# Autodesk Inventor assembly: korp
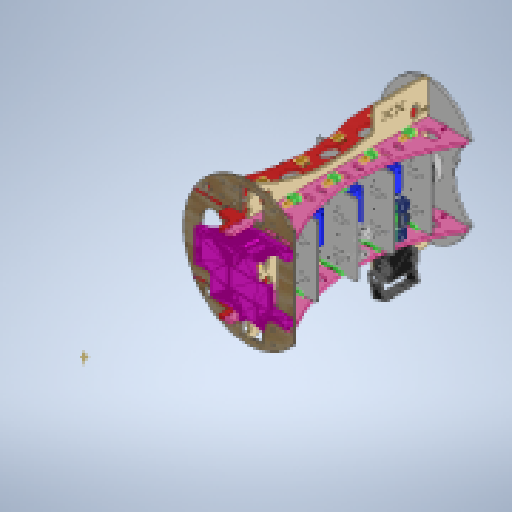
[picture p0: Inventor's stored thumbnail of the model, 512x512]
Saved by Autodesk Inventor 2023.1 (Build 271208000, 208)
## iProperties
Created: 2023-03-13
Part Number: korp
Document SubType Name: Assembly
Designer: User
Author: User
## Documents named in this file (23)
- C:\Users\DELL\reposGitHub\Cheburashka\Cheburashka_construction\korpus\korp.iam
- C:\Users\DELL\reposGitHub\Cheburashka\Cheburashka_construction\korpus\нижний эллипс тела.ipt
- C:\Users\DELL\reposGitHub\Cheburashka\Cheburashka_construction\korpus\грань тела.ipt
- C:\Users\DELL\reposGitHub\Cheburashka\Cheburashka_construction\korpus\Servo.ipt
- C:\Users\DELL\reposGitHub\Cheburashka\Cheburashka_construction\platform\KRAVT_holder_2 (1).ipt
- C:\Users\DELL\reposGitHub\Cheburashka\Cheburashka_construction\korpus\ребро.ipt
- C:\Users\DELL\reposGitHub\Cheburashka\Cheburashka_construction\korpus\ребро_MIR.ipt
- C:\Users\DELL\reposGitHub\Cheburashka\Cheburashka_construction\korpus\креп.ipt
- C:\Users\DELL\reposGitHub\Cheburashka\Cheburashka_construction\korpus\ребро0.5.ipt
- C:\Users\DELL\reposGitHub\Cheburashka\Cheburashka_construction\korpus\стабилизатор.ipt
- C:\Users\DELL\reposGitHub\Cheburashka\Cheburashka_construction\korpus\ограничитель.ipt
- C:\Users\DELL\reposGitHub\Cheburashka\Cheburashka_construction\korpus\ребро0.5_MIR3.ipt
- C:\Users\DELL\reposGitHub\Cheburashka\Cheburashka_construction\korpus\фанера.ipt
- C:\Users\DELL\reposGitHub\Cheburashka\Cheburashka_construction\korpus\ограничитель_MIR.ipt
- C:\Users\DELL\reposGitHub\Cheburashka\Cheburashka_construction\korpus\палка.ipt
- C:\Users\DELL\reposGitHub\Cheburashka\Cheburashka_construction\korpus\креп_MIR2.ipt
- C:\Users\DELL\reposGitHub\Cheburashka\Cheburashka_construction\korpus\палка_MIR.ipt
- C:\Users\DELL\reposGitHub\Cheburashka\Cheburashka_construction\korpus\raspberry-pi-4-model-b-1.snapshot.3\Raspberry Pi 4 Model B.iam
- C:\Users\DELL\reposGitHub\Cheburashka\Cheburashka_construction\korpus\arduino-mega-2650-1.snapshot.2\arduino MEGA2650.iam
- C:\Users\DELL\reposGitHub\Cheburashka\Cheburashka_construction\korpus\acc2.ipt
- C:\Users\DELL\reposGitHub\Cheburashka\Cheburashka_construction\korpus\acc1.ipt
- C:\Users\DELL\reposGitHub\Cheburashka\Cheburashka_construction\face\лицо\креп_сервы.ipt
- C:\Users\DELL\reposGitHub\Cheburashka\Cheburashka_construction\korpus\turn.iam
## Components (54 placed, 22 different names)
1. нижний эллипс тела:1 — Совмещение:100, Совмещение:121, Совмещение:139, Совмещение:140, Совмещение:209, Совмещение:210
2. грань тела:1 — Совмещение:209, Совмещение:210, Совмещение:211, Совмещение:214, Совмещение:224, Совмещение:225, Совмещение:229, Совмещение:308
3. KRAVT_holder_2 (1):1 — Совмещение:100
4. ребро:1 — Совмещение:184, Совмещение:264, Совмещение:307
5. ребро_MIR:1 — Совмещение:122, Совмещение:188, Совмещение:204, Совмещение:305
6. креп:1 — Совмещение:159, Совмещение:166, Совмещение:221, Совмещение:222
7. креп:2 — Совмещение:164, Совмещение:165
8. креп:3 — Совмещение:162, Совмещение:163
9. креп:4 — Совмещение:160, Совмещение:161, Совмещение:219, Совмещение:220
10. креп:5 — Совмещение:167, Совмещение:168
11. креп:6 — Совмещение:169, Совмещение:170, Совмещение:183, Совмещение:217, Совмещение:218
12. креп:7 — Совмещение:261, Совмещение:262, Совмещение:265, Совмещение:266
13. креп:8 — Совмещение:171, Совмещение:172
14. ребро0.5:1 — Совмещение:121, Совмещение:122, Совмещение:126, Совмещение:128, Совмещение:129, Совмещение:130, Совмещение:132, Совмещение:133, Совмещение:135, Совмещение:136, Совмещение:138, Совмещение:186, Совмещение:187, Совмещение:189, Совмещение:190, Совмещение:191, Совмещение:192, Совмещение:193, Совмещение:194, Совмещение:195, Совмещение:196, Совмещение:197, Совмещение:198, Совмещение:199, Совмещение:200, Совмещение:201, Совмещение:202
15. стабилизатор:1
16. ребро0.5_MIR3:1 — Совмещение:139, Совмещение:140, Совмещение:159, Совмещение:160, Совмещение:161, Совмещение:162, Совмещение:163, Совмещение:164, Совмещение:165, Совмещение:166, Совмещение:167, Совмещение:168, Совмещение:169, Совмещение:170, Совмещение:171, Совмещение:172, Совмещение:261, Совмещение:262
17. ограничитель:1 — Совмещение:126, Совмещение:128, Совмещение:129
18. ограничитель:2 — Совмещение:130, Совмещение:132
19. ограничитель:3 — Совмещение:133, Совмещение:135
20. ограничитель:4 — Совмещение:136, Совмещение:138
21. фанера:1 — Совмещение:305, Совмещение:306
22. ограничитель_MIR:1
23. ограничитель_MIR:2
24. ограничитель_MIR:3
25. ограничитель_MIR:4
26. палка:1 — Совмещение:264, Совмещение:265, Совмещение:266
27. креп_MIR2:1 — Совмещение:199, Совмещение:200, Совмещение:203, Совмещение:303, Совмещение:304
28. креп_MIR2:2 — Совмещение:201, Совмещение:202
29. креп_MIR2:3 — Совмещение:197, Совмещение:198
30. креп_MIR2:4 — Совмещение:185, Совмещение:186, Совмещение:187, Совмещение:301, Совмещение:302
31. креп_MIR2:5 — Совмещение:195, Совмещение:196
32. креп_MIR2:6 — Совмещение:189, Совмещение:190, Совмещение:299, Совмещение:300
33. креп_MIR2:7 — Совмещение:180, Совмещение:181, Совмещение:182, Совмещение:191, Совмещение:192, Совмещение:306
34. креп_MIR2:8 — Совмещение:193, Совмещение:194
35. палка_MIR:1 — Совмещение:180, Совмещение:181, Совмещение:182
36. фанера:2 — Совмещение:183, Совмещение:184, Совмещение:212, Совмещение:213
37. фанера:3 — Совмещение:203, Совмещение:204
38. фанера:4 — Совмещение:185, Совмещение:188, Совмещение:215, Совмещение:216
39. Raspberry Pi 4 Model B:1 [sub-assembly] — Совмещение:212, Совмещение:213
40. arduino MEGA2650:1 [sub-assembly] — Совмещение:215, Совмещение:216
41. стабилизатор:2 — Совмещение:214
42. стабилизатор:3 — Совмещение:211
43. палка:2 — Совмещение:219, Совмещение:220
44. палка:3 — Совмещение:221, Совмещение:222
45. палка:4 — Совмещение:217, Совмещение:218
46. Servo:5 — Совмещение:224, Совмещение:225, Совмещение:227, Совмещение:228
47. acc2:1 — Совмещение:227, Совмещение:228
48. acc1:1 — Совмещение:229
49. креп_сервы:1
50. креп_сервы:2
51. палка_MIR:2 — Совмещение:299, Совмещение:300
52. палка_MIR:3 — Совмещение:301, Совмещение:302
53. палка_MIR:4 — Совмещение:303, Совмещение:304
54. turn:1 [sub-assembly] — Совмещение:307, Совмещение:308
## Relationships (88: Mate 87, Angle 1)
- Совмещение:100 [Mate]: нижний эллипс тела:1 ↔ KRAVT_holder_2 (1):1
- Совмещение:121 [Mate]: нижний эллипс тела:1 ↔ ребро0.5:1
- Совмещение:122 [Mate]: ребро_MIR:1 ↔ ребро0.5:1
- Совмещение:126 [Mate]: ребро0.5:1 ↔ ограничитель:1
- Совмещение:128 [Mate]: ребро0.5:1 ↔ ограничитель:1
- Совмещение:129 [Mate]: ребро0.5:1 ↔ ограничитель:1
- Совмещение:130 [Mate]: ребро0.5:1 ↔ ограничитель:2
- Совмещение:132 [Mate]: ребро0.5:1 ↔ ограничитель:2
- Совмещение:133 [Mate]: ребро0.5:1 ↔ ограничитель:3
- Совмещение:135 [Mate]: ребро0.5:1 ↔ ограничитель:3
- Совмещение:136 [Mate]: ребро0.5:1 ↔ ограничитель:4
- Совмещение:138 [Mate]: ребро0.5:1 ↔ ограничитель:4
- Совмещение:139 [Mate]: нижний эллипс тела:1 ↔ ребро0.5_MIR3:1
- Совмещение:140 [Mate]: нижний эллипс тела:1 ↔ ребро0.5_MIR3:1
- Совмещение:159 [Mate]: креп:1 ↔ ребро0.5_MIR3:1
- Совмещение:160 [Mate]: креп:4 ↔ ребро0.5_MIR3:1
- Совмещение:161 [Mate]: креп:4 ↔ ребро0.5_MIR3:1
- Совмещение:162 [Mate]: креп:3 ↔ ребро0.5_MIR3:1
- Совмещение:163 [Mate]: креп:3 ↔ ребро0.5_MIR3:1
- Совмещение:164 [Mate]: креп:2 ↔ ребро0.5_MIR3:1
- Совмещение:165 [Mate]: креп:2 ↔ ребро0.5_MIR3:1
- Совмещение:166 [Mate]: креп:1 ↔ ребро0.5_MIR3:1
- Совмещение:167 [Mate]: креп:5 ↔ ребро0.5_MIR3:1
- Совмещение:168 [Mate]: креп:5 ↔ ребро0.5_MIR3:1
- Совмещение:169 [Mate]: креп:6 ↔ ребро0.5_MIR3:1
- Совмещение:170 [Mate]: креп:6 ↔ ребро0.5_MIR3:1
- Совмещение:171 [Mate]: креп:8 ↔ ребро0.5_MIR3:1
- Совмещение:172 [Mate]: креп:8 ↔ ребро0.5_MIR3:1
- Совмещение:180 [Mate]: креп_MIR2:7 ↔ палка_MIR:1
- Совмещение:181 [Mate]: креп_MIR2:7 ↔ палка_MIR:1
- Совмещение:182 [Mate]: креп_MIR2:7 ↔ палка_MIR:1
- Совмещение:183 [Mate]: креп:6 ↔ фанера:2
- Совмещение:184 [Mate]: ребро:1 ↔ фанера:2
- Совмещение:185 [Mate]: креп_MIR2:4 ↔ фанера:4
- Совмещение:186 [Mate]: ребро0.5:1 ↔ креп_MIR2:4
- Совмещение:187 [Mate]: ребро0.5:1 ↔ креп_MIR2:4
- Совмещение:188 [Mate]: ребро_MIR:1 ↔ фанера:4
- Совмещение:189 [Mate]: ребро0.5:1 ↔ креп_MIR2:6
- Совмещение:190 [Mate]: ребро0.5:1 ↔ креп_MIR2:6
- Совмещение:191 [Mate]: ребро0.5:1 ↔ креп_MIR2:7
- Совмещение:192 [Mate]: ребро0.5:1 ↔ креп_MIR2:7
- Совмещение:193 [Mate]: ребро0.5:1 ↔ креп_MIR2:8
- Совмещение:194 [Mate]: ребро0.5:1 ↔ креп_MIR2:8
- Совмещение:195 [Mate]: ребро0.5:1 ↔ креп_MIR2:5
- Совмещение:196 [Mate]: ребро0.5:1 ↔ креп_MIR2:5
- Совмещение:197 [Mate]: ребро0.5:1 ↔ креп_MIR2:3
- Совмещение:198 [Mate]: ребро0.5:1 ↔ креп_MIR2:3
- Совмещение:199 [Mate]: ребро0.5:1 ↔ креп_MIR2:1
- Совмещение:200 [Mate]: ребро0.5:1 ↔ креп_MIR2:1
- Совмещение:201 [Mate]: ребро0.5:1 ↔ креп_MIR2:2
- Совмещение:202 [Mate]: ребро0.5:1 ↔ креп_MIR2:2
- Совмещение:203 [Mate]: креп_MIR2:1 ↔ фанера:3
- Совмещение:204 [Mate]: ребро_MIR:1 ↔ фанера:3
- Совмещение:209 [Mate]: нижний эллипс тела:1 ↔ грань тела:1
- Совмещение:210 [Mate]: нижний эллипс тела:1 ↔ грань тела:1
- Совмещение:211 [Mate]: грань тела:1 ↔ стабилизатор:3
- Совмещение:212 [Mate]: фанера:2 ↔ Raspberry Pi 4 Model B:1
- Совмещение:213 [Mate]: фанера:2 ↔ Raspberry Pi 4 Model B:1
- Совмещение:214 [Mate]: грань тела:1 ↔ стабилизатор:2
- Совмещение:215 [Mate]: фанера:4 ↔ arduino MEGA2650:1
- Совмещение:216 [Mate]: фанера:4 ↔ arduino MEGA2650:1
- Совмещение:217 [Mate]: креп:6 ↔ палка:4
- Совмещение:218 [Mate]: креп:6 ↔ палка:4
- Совмещение:219 [Mate]: креп:4 ↔ палка:2
- Совмещение:220 [Mate]: креп:4 ↔ палка:2
- Совмещение:221 [Mate]: креп:1 ↔ палка:3
- Совмещение:222 [Mate]: креп:1 ↔ палка:3
- Совмещение:224 [Mate]: грань тела:1 ↔ Servo:5
- Совмещение:225 [Mate]: грань тела:1 ↔ Servo:5
- Совмещение:227 [Mate]: Servo:5 ↔ acc2:1
- Совмещение:228 [Mate]: Servo:5 ↔ acc2:1
- Совмещение:229 [Mate]: грань тела:1 ↔ acc1:1
- Угол:1 [Angle] (0 deg)
- Совмещение:261 [Mate]: креп:7 ↔ ребро0.5_MIR3:1
- Совмещение:262 [Mate]: креп:7 ↔ ребро0.5_MIR3:1
- Совмещение:264 [Mate]: ребро:1 ↔ палка:1
- Совмещение:265 [Mate]: креп:7 ↔ палка:1
- Совмещение:266 [Mate]: креп:7 ↔ палка:1
- Совмещение:299 [Mate]: креп_MIR2:6 ↔ палка_MIR:2
- Совмещение:300 [Mate]: креп_MIR2:6 ↔ палка_MIR:2
- Совмещение:301 [Mate]: креп_MIR2:4 ↔ палка_MIR:3
- Совмещение:302 [Mate]: креп_MIR2:4 ↔ палка_MIR:3
- Совмещение:303 [Mate]: креп_MIR2:1 ↔ палка_MIR:4
- Совмещение:304 [Mate]: креп_MIR2:1 ↔ палка_MIR:4
- Совмещение:305 [Mate]: ребро_MIR:1 ↔ фанера:1
- Совмещение:306 [Mate]: фанера:1 ↔ креп_MIR2:7
- Совмещение:307 [Mate]: ребро:1 ↔ turn:1
- Совмещение:308 [Mate]: грань тела:1 ↔ turn:1
